# Autodesk Inventor assembly: Full Robot Arm
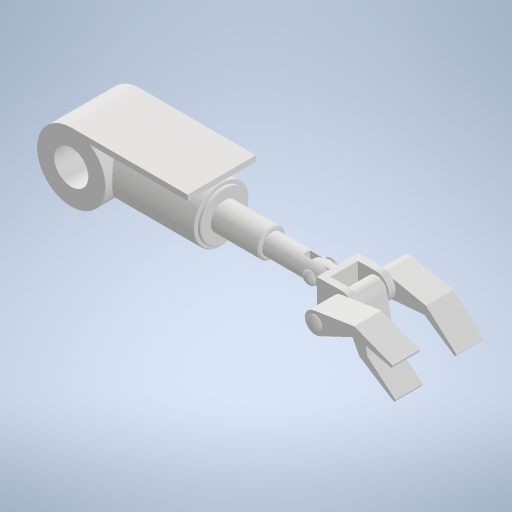
[picture p0: Inventor's stored thumbnail of the model, 512x512]
Saved by Autodesk Inventor 2024 (Build 280153000, 153)
## iProperties
Created: 2023-06-06
Part Number: Full Robot Arm
Document SubType Name: Assembly
Designer: vilas
Author: vilas
## Documents named in this file (6)
- D:\Parth Folder\ES101\Project\Full Robot Arm.iam
- D:\Parth Folder\ES101\Project\Hydraulic Arm.ipt
- D:\Parth Folder\ES101\Project\Claw Palm.ipt
- D:\Parth Folder\ES101\Project\Claw.ipt
- D:\Parth Folder\ES101\Project\Axis(1).ipt
- D:\Parth Folder\ES101\Project\Axis(2).ipt
## Components (7 placed, 5 different names)
1. Hydraulic Arm:1 — Mate:2, Mate:11, Mate:13
2. Claw Palm:1 — Mate:2, Mate:3, Mate:4, Mate:5, Mate:6, Mate:7, Mate:8, Mate:12, Mate:13
3. Claw:1 — Mate:7, Mate:8
4. Claw:2 — Mate:5, Mate:6, Mate:9, Mate:10
5. Claw:3 — Mate:3, Mate:4
6. Axis(1):1 — Mate:9, Mate:10
7. Axis(2):1 — Mate:11, Mate:12
## Relationships (12: Mate 12)
- Mate:2: Hydraulic Arm:1 ↔ Claw Palm:1
- Mate:3: Claw Palm:1 ↔ Claw:3
- Mate:4: Claw Palm:1 ↔ Claw:3
- Mate:5: Claw Palm:1 ↔ Claw:2
- Mate:6: Claw Palm:1 ↔ Claw:2
- Mate:7: Claw Palm:1 ↔ Claw:1
- Mate:8: Claw Palm:1 ↔ Claw:1
- Mate:9: Claw:2 ↔ Axis(1):1
- Mate:10: Claw:2 ↔ Axis(1):1
- Mate:11: Hydraulic Arm:1 ↔ Axis(2):1
- Mate:12 (5 mm): Claw Palm:1 ↔ Axis(2):1
- Mate:13: Hydraulic Arm:1 ↔ Claw Palm:1
